# Autodesk Inventor assembly: DIY TableSaw
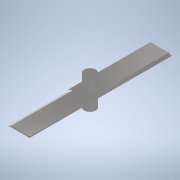
[picture p0: Inventor's stored thumbnail of the model, 180x180]
Saved by Autodesk Inventor 2022 (Build 260153000, 153)
## iProperties
Created: 2022-07-28
Part Number: DIY TableSaw
Document SubType Name: Assembly
Designer: Nathan Cai
Author: Nathan Cai
## Documents named in this file (3)
- C:\Users\Nathan Cai\Documents\Inventor\Asorted Parts\DIY Tablesaw Parts\DIY TableSaw.iam
- C:\Users\Nathan Cai\Documents\Inventor\Asorted Parts\DIY Tablesaw Parts\DIY TableSaw - BLADE.ipt
- C:\Users\Nathan Cai\Documents\Inventor\Asorted Parts\DIY Tablesaw Parts\HUB.ipt
## Components (2 placed, 2 different names)
1. DIY TableSaw - BLADE:1 — Mate:1, Flush:1
2. HUB:1 — Mate:1, Flush:1
## Relationships (2: Mate 1, Flush 1)
- Mate:1: DIY TableSaw - BLADE:1 ↔ HUB:1
- Flush:1 (-20 mm): DIY TableSaw - BLADE:1 ↔ HUB:1
